# Autodesk Inventor assembly: CP675
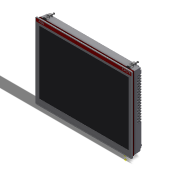
[picture p0: Inventor's stored thumbnail of the model, 180x180]
Saved by Autodesk Inventor 2015 (Build 190159000, 159)
## iProperties
Created: 2014-04-07
Part Number: CP675
Document SubType Name: Assembly
Designer: alid
Description: HMI PANEL CP600 series
Vendor: ABB
Author: alid
## Documents named in this file (5)
- C:\Vault Workspace\Inventor2015new\Projects\Electrical Components\PLCIO\ABB\CP675\ABB_CP675_PANEL.IAM
- C:\Vault Workspace\Inventor2015new\Projects\Electrical Components\PLCIO\ABB\CP675\ABB_CP675_Panel.ipt
- C:\Vault Workspace\Inventor2015new\Projects\Electrical Components\PLCIO\ABB\CP675\CP675 Fixing.iam
- C:\Vault Workspace\Inventor2015new\Projects\7_Electrical\HMI-Panel Components\PLC-Conn-F.ipt
- C:\Vault Workspace\Inventor2015new\Projects\7_Electrical\HMI-Panel Components\PLC-Conn-M.ipt
## Components (7 placed, 4 different names)
1. ABB_CP675_Panel:1 — Rigid:2, Rigid:3, Rigid:4, Rigid:5
2. CP675 Fixing:1 [sub-assembly]
3. CP675 Fixing:2 [sub-assembly] — Rigid:2
4. CP675 Fixing:3 [sub-assembly] — Rigid:4
5. CP675 Fixing:4 [sub-assembly] — Rigid:3
6. PLC-Conn-F:1 — Rigid:5, Rigid:6
7. PLC-Conn-M:1 — Rigid:6
## Relationships (7: WeldJoint 6, Angle 1)
- [WeldJoint]: ABB_CP675_Panel:1 ↔ CP675 Fixing:1
- [Angle] (180 deg): ABB_CP675_Panel:1 ↔ CP675 Fixing:1
- Rigid:2 [WeldJoint]: ABB_CP675_Panel:1 ↔ CP675 Fixing:2
- Rigid:3 [WeldJoint]: ABB_CP675_Panel:1 ↔ CP675 Fixing:4
- Rigid:4 [WeldJoint]: ABB_CP675_Panel:1 ↔ CP675 Fixing:3
- Rigid:5 [WeldJoint]: ABB_CP675_Panel:1 ↔ PLC-Conn-F:1
- Rigid:6 [WeldJoint]: PLC-Conn-F:1 ↔ PLC-Conn-M:1
